# Autodesk Inventor assembly: dual_motor_testbed_cover
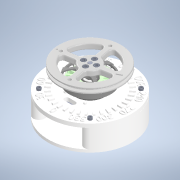
[picture p0: Inventor's stored thumbnail of the model, 180x180]
Saved by Autodesk Inventor 2022.2 (Build 262287000, 287)
## iProperties
Created: 2020-06-08
Part Number: dual_motor_testbed_cover
Document SubType Name: Assembly
Designer: Jochen
Sending System: SolidWorks 2017
Last Author: Felix
Last Saved: 2021-02-24
Author: Jochen
## Documents named in this file (5)
- D:\Projects\Chewbacca\CAD\Tools\Motor Testbed\MotorTestbed.iam
- D:\Projects\Chewbacca\CAD\Tools\Motor Testbed\MotorTestBedScaffold.ipt
- D:\Projects\Chewbacca\CAD\Tools\Motor Testbed\encoder_avago_aedt_9810.iam
- D:\Projects\Chewbacca\CAD\Tools\Motor Testbed\fastener_shcs_m2.5_8.ipt
- D:\Projects\Chewbacca\CAD\Tools\Motor Testbed\MotorModuleTest.iam
## Components (7 placed, 4 different names)
1. dual_motor_testbed_cover:1 — Mate:1, Mate:5, Mate:6, Mate:7, Mate:8, Mate:14, Mate:15, Mate:16, Mate:17
2. encoder_avago_aedt_9810:1 [sub-assembly] — Mate:5, Mate:6
3. fastener_shcs_m2.5_8:3 — Mate:14
4. fastener_shcs_m2.5_8:4 — Mate:16
5. fastener_shcs_m2.5_8:7 — Mate:15
6. fastener_shcs_m2.5_8:8 — Mate:17
7. motor_module:2 [sub-assembly] — Mate:1, Mate:7, Mate:8
## Relationships (9: Mate 9)
- Mate:1: dual_motor_testbed_cover:1 ↔ motor_module:2
- Mate:5: dual_motor_testbed_cover:1 ↔ encoder_avago_aedt_9810:1
- Mate:6: dual_motor_testbed_cover:1 ↔ encoder_avago_aedt_9810:1
- Mate:7: dual_motor_testbed_cover:1 ↔ motor_module:2
- Mate:8: dual_motor_testbed_cover:1 ↔ motor_module:2
- Mate:14: dual_motor_testbed_cover:1 ↔ fastener_shcs_m2.5_8:3
- Mate:15: dual_motor_testbed_cover:1 ↔ fastener_shcs_m2.5_8:7
- Mate:16: dual_motor_testbed_cover:1 ↔ fastener_shcs_m2.5_8:4
- Mate:17: dual_motor_testbed_cover:1 ↔ fastener_shcs_m2.5_8:8
